# Autodesk Inventor assembly: Ribbon_Twitter1
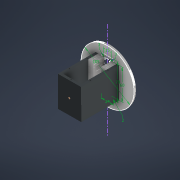
[picture p0: Inventor's stored thumbnail of the model, 180x180]
Saved by Autodesk Inventor 2022 (Build 260153070, 153G)
## iProperties
Created: 2022-02-03
Part Number: Ribbon_Twitter1
Document SubType Name: Assembly
Designer: kalugin_a
Author: kalugin_a
## Documents named in this file (4)
- C:\Users\kalugin_a\Documents\Inventor\TUTO\MELAS\Workspace\Ribbon_Twitter1.iam
- C:\Users\kalugin_a\Documents\Inventor\TUTO\MELAS\Workspace\фланец2.ipt
- C:\Users\kalugin_a\Documents\Inventor\TUTO\MELAS\Workspace\magnetGuide.ipt
- C:\Users\kalugin_a\Documents\Inventor\TUTO\MELAS\Workspace\Magnit.ipt
## Components (4 placed, 3 different names)
1. magnetGuide:1 — Совмещение:7, Совмещение:8, Совмещение:9, Совмещение:10
2. фланец2:1 — Совмещение:4, Совмещение:6, Совмещение:7, Совмещение:8
3. Magnit:1 — Совмещение:6, Совмещение:9
4. Magnit:2 — Совмещение:4, Совмещение:10
## Relationships (6: Mate 6)
- Совмещение:4 [Mate]: фланец2:1 ↔ Magnit:2
- Совмещение:6 [Mate]: фланец2:1 ↔ Magnit:1
- Совмещение:7 [Mate]: magnetGuide:1 ↔ фланец2:1
- Совмещение:8 [Mate]: magnetGuide:1 ↔ фланец2:1
- Совмещение:9 [Mate]: magnetGuide:1 ↔ Magnit:1
- Совмещение:10 [Mate]: magnetGuide:1 ↔ Magnit:2
